# Autodesk Inventor assembly: NanoSumo_part1
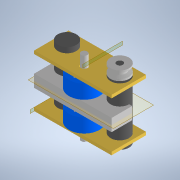
[picture p0: Inventor's stored thumbnail of the model, 180x180]
Saved by Autodesk Inventor 2022.3 (Build 263350000, 350)
## iProperties
Created: 2022-12-14
Part Number: NanoSumo_part1
Document SubType Name: Assembly
Designer: komputer
Author: komputer
## Documents named in this file (7)
- C:\Users\komputer\Documents\Inventor\NanoSumo\NanoSumo_part1.iam
- C:\Users\komputer\Documents\Inventor\NanoSumo\silnik.ipt
- C:\Users\komputer\Documents\Inventor\NanoSumo\bok.ipt
- C:\Users\komputer\Documents\Inventor\NanoSumo\kółko.ipt
- C:\Users\komputer\Documents\Inventor\NanoSumo\srodek.ipt
- C:\Users\komputer\Documents\Inventor\NanoSumo\kolo.ipt
- C:\Users\komputer\Documents\Inventor\NanoSumo\oponka.ipt
## Components (11 placed, 6 different names)
1. silnik:1 — Mate:2, Flush:2, Mate:3, Mate:6, Mate:7, Flush:6
2. silnik:2 — Flush:1, Mate:1, Mate:4, Flush:3, Flush:8
3. bok:1 — Mate:2, Flush:2, Mate:4, Mate:5
4. bok:2 — Flush:1, Mate:1, Mate:3, Mate:5, Flush:4, Flush:5, Mate:8
5. kółko:1 — Flush:3, Flush:4
6. kółko:2 — Mate:6, Mate:7
7. srodek:1 — Flush:5
8. kolo:1 — Flush:6, Flush:7
9. oponka:1 — Flush:7
10. oponka:2 — Mate:9, Mate:10
11. kolo:2 — Flush:8, Mate:8, Mate:9, Mate:10
## Relationships (18: Mate 10, Flush 8)
- Flush:1: silnik:2 ↔ bok:2
- Mate:1: silnik:2 ↔ bok:2
- Mate:2: silnik:1 ↔ bok:1
- Flush:2: silnik:1 ↔ bok:1
- Mate:3: silnik:1 ↔ bok:2
- Mate:4: silnik:2 ↔ bok:1
- Mate:5 (15 mm): bok:1 ↔ bok:2
- Flush:3: silnik:2 ↔ kółko:1
- Flush:4: bok:2 ↔ kółko:1
- Mate:6: silnik:1 ↔ kółko:2
- Mate:7: silnik:1 ↔ kółko:2
- Flush:5 (7.5 mm): bok:2 ↔ srodek:1
- Flush:6: silnik:1 ↔ kolo:1
- Flush:7: kolo:1 ↔ oponka:1
- Flush:8: silnik:2 ↔ kolo:2
- Mate:8: bok:2 ↔ kolo:2
- Mate:9: oponka:2 ↔ kolo:2
- Mate:10: oponka:2 ↔ kolo:2
